# Autodesk Inventor assembly: HVU_sample_chamber_half
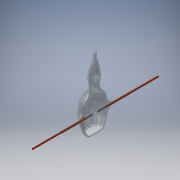
[picture p0: Inventor's stored thumbnail of the model, 180x180]
Saved by Autodesk Inventor 2017 (Build 210142000, 142)
## iProperties
Part Number: HVU_sample_chamber_half
Material: Generisch
Document SubType Name: Assembly
Designer: David Merges
Author: David Merges
## Documents named in this file (7)
- C:\Seafile\Meine Bibliothek\Inventor\EXCISS\2019\HVU_sample_chamber_half.iam
- C:\Seafile\Meine Bibliothek\Inventor\EXCISS\2019\HVU_elekrode_tip_r.ipt
- C:\Seafile\Meine Bibliothek\Inventor\EXCISS\2019\HVU_elekrode_tip_t.ipt
- C:\Seafile\Meine Bibliothek\Inventor\EXCISS\2019\HVU_spark.ipt
- C:\Seafile\Meine Bibliothek\Inventor\EXCISS\2019\HVU_elektrode_Cu.ipt
- C:\Seafile\Meine Bibliothek\Inventor\EXCISS\2019\HVU_dust.ipt
- C:\Seafile\Meine Bibliothek\Inventor\EXCISS\2019\HVU_sample_chamber_half.ipt
## Components (164 placed, 6 different names)
1. HVU_elekrode_tip_r:1 — Passend:8, Fluchtend:2, Passend:11, Passend:14
2. HVU_elekrode_tip_t:1 — Passend:9, Passend:10, Passend:12, Passend:13
3. HVU_spark:1 — Fluchtend:1
4. HVU_sample_chamber_half:1 — Fluchtend:4, Passend:17
5. HVU_elektrode_Cu:1 — Passend:12, Passend:13
6. HVU_elektrode_Cu:2 — Passend:11, Passend:14, Passend:17
7. HVU_dust:1
8. HVU_dust:2
9. HVU_dust:3
10. HVU_dust:4
11. HVU_dust:5
12. HVU_dust:6
13. HVU_dust:7
14. HVU_dust:8
15. HVU_dust:9
16. HVU_dust:10
17. HVU_dust:11
18. HVU_dust:12
19. HVU_dust:13
20. HVU_dust:14
21. HVU_dust:15
22. HVU_dust:16
23. HVU_dust:17
24. HVU_dust:18
25. HVU_dust:19
26. HVU_dust:20
27. HVU_dust:21
28. HVU_dust:22
29. HVU_dust:23
30. HVU_dust:24
31. HVU_dust:25
32. HVU_dust:26
33. HVU_dust:27
34. HVU_dust:28
35. HVU_dust:29
36. HVU_dust:30
37. HVU_dust:31
38. HVU_dust:32
39. HVU_dust:33
40. HVU_dust:34
41. HVU_dust:35
42. HVU_dust:36
43. HVU_dust:37
44. HVU_dust:38
45. HVU_dust:39
46. HVU_dust:40
47. HVU_dust:41
48. HVU_dust:42
49. HVU_dust:43
50. HVU_dust:44
51. HVU_dust:45
52. HVU_dust:46
53. HVU_dust:47
54. HVU_dust:48
55. HVU_dust:49
56. HVU_dust:50
57. HVU_dust:51
58. HVU_dust:52
59. HVU_dust:53
60. HVU_dust:54
61. HVU_dust:55
62. HVU_dust:56
63. HVU_dust:57
64. HVU_dust:58
65. HVU_dust:59
66. HVU_dust:60
67. HVU_dust:61
68. HVU_dust:62
69. HVU_dust:63
70. HVU_dust:64
71. HVU_dust:65
72. HVU_dust:66
73. HVU_dust:67
74. HVU_dust:68
75. HVU_dust:69
76. HVU_dust:70
77. HVU_dust:71
78. HVU_dust:72
79. HVU_dust:73
80. HVU_dust:74
81. HVU_dust:75
82. HVU_dust:76
83. HVU_dust:77
84. HVU_dust:78
85. HVU_dust:79
86. HVU_dust:80
87. HVU_dust:81
88. HVU_dust:82
89. HVU_dust:83
90. HVU_dust:84
91. HVU_dust:85
92. HVU_dust:86
93. HVU_dust:87
94. HVU_dust:88
95. HVU_dust:89
96. HVU_dust:90
97. HVU_dust:91
98. HVU_dust:92
99. HVU_dust:93
100. HVU_dust:94
101. HVU_dust:95
102. HVU_dust:96
103. HVU_dust:97
104. HVU_dust:98
105. HVU_dust:99
106. HVU_dust:100
107. HVU_dust:101
108. HVU_dust:102
109. HVU_dust:103
110. HVU_dust:104
111. HVU_dust:105
112. HVU_dust:106
113. HVU_dust:107
114. HVU_dust:108
115. HVU_dust:109
116. HVU_dust:110
117. HVU_dust:111
118. HVU_dust:112
119. HVU_dust:113
120. HVU_dust:114
121. HVU_dust:115
122. HVU_dust:116
123. HVU_dust:117
124. HVU_dust:118
125. HVU_dust:119
126. HVU_dust:120
127. HVU_dust:121
128. HVU_dust:122
129. HVU_dust:123
130. HVU_dust:124
131. HVU_dust:125
132. HVU_dust:126
133. HVU_dust:127
134. HVU_dust:128
135. HVU_dust:129
136. HVU_dust:130
137. HVU_dust:131
138. HVU_dust:132
139. HVU_dust:133
140. HVU_dust:134
141. HVU_dust:135
142. HVU_dust:136
143. HVU_dust:137
144. HVU_dust:138
145. HVU_dust:139
146. HVU_dust:140
147. HVU_dust:141
148. HVU_dust:142
149. HVU_dust:143
150. HVU_dust:144
151. HVU_dust:145
152. HVU_dust:146
153. HVU_dust:147
154. HVU_dust:148
155. HVU_dust:149
156. HVU_dust:150
157. HVU_dust:151
158. HVU_dust:152
159. HVU_dust:153
160. HVU_dust:154
161. HVU_dust:155
162. HVU_dust:156
163. HVU_dust:157
164. HVU_dust:158
## Relationships (11: Mate 8, Flush 3)
- Fluchtend:1 [Flush]: HVU_spark:1
- Passend:8 [Mate]: HVU_elekrode_tip_r:1
- Passend:9 [Mate]: HVU_elekrode_tip_t:1
- Passend:10 [Mate] (-1.25 mm): HVU_elekrode_tip_t:1
- Fluchtend:2 [Flush] (-1.25 mm): HVU_elekrode_tip_r:1
- Passend:11 [Mate]: HVU_elekrode_tip_r:1 ↔ HVU_elektrode_Cu:2
- Passend:12 [Mate]: HVU_elekrode_tip_t:1 ↔ HVU_elektrode_Cu:1
- Passend:13 [Mate]: HVU_elekrode_tip_t:1 ↔ HVU_elektrode_Cu:1
- Passend:14 [Mate]: HVU_elekrode_tip_r:1 ↔ HVU_elektrode_Cu:2
- Fluchtend:4 [Flush]: HVU_sample_chamber_half:1
- Passend:17 [Mate]: HVU_sample_chamber_half:1 ↔ HVU_elektrode_Cu:2
